# Autodesk Inventor assembly: Holder
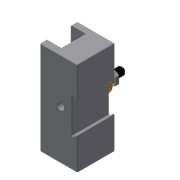
[picture p0: Inventor's stored thumbnail of the model, 180x180]
Saved by Autodesk Inventor 2016 (Build 200138000, 138)
## iProperties
Created: 2020-10-21
Part Number: Holder
Document SubType Name: Assembly
Designer: extract
Author: extract
## Documents named in this file (5)
- D:\GDrive\Proyecto_Torno\Tool_post\Holder.iam
- D:\GDrive\Proyecto_Torno\Tool_post\Turning and Facing Holder.ipt
- D:\GDrive\Proyecto_Torno\Tool_post\Press.ipt
- D:\GDrive\Proyecto_Torno\Tool_post\hex.ipt
- D:\GDrive\Proyecto_Torno\Tool_post\thread.ipt
## Components (4 placed, 4 different names)
1. Turning and Facing Holder:1
2. Press:1
3. hex:1
4. thread:1
## Relationships (3: Insert 2, CylindricalJoint 1)
- [Insert]: Turning and Facing Holder:1 ↔ Press:1
- [Insert]: Press:1 ↔ hex:1
- [CylindricalJoint]: hex:1 ↔ thread:1
